# Autodesk Inventor assembly: axis5_6  compact
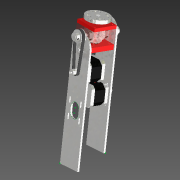
[picture p0: Inventor's stored thumbnail of the model, 180x180]
Saved by Autodesk Inventor 2020 (Build 240168000, 168)
## iProperties
Created: 2020-05-15
Part Number: axis5_6  compact
Document SubType Name: Assembly
Designer: stefa
Author: stefa
## Documents named in this file (9)
- D:\github_gedeeld\BeerMinder\3D-model\axis5_6\axis5_6  compact.iam
- D:\github_gedeeld\BeerMinder\3D-model\pulleys\GT2 Timing Pulley 36T - 8mm as.ipt
- D:\github_gedeeld\BeerMinder\3D-model\stepper motors\42BYG Stepper Motor.ipt
- D:\github_gedeeld\BeerMinder\3D-model\pulleys\GT2 Pulley 16T - 5mm as.ipt
- D:\github_gedeeld\BeerMinder\3D-model\axis5_6\bovenarm - links.ipt
- D:\github_gedeeld\BeerMinder\3D-model\bearings\lager 8mm - buiten 14 (sven 2 stuks).ipt
- D:\github_gedeeld\BeerMinder\3D-model\axis5_6\differential gearbox compact.iam
- D:\github_gedeeld\BeerMinder\3D-model\pulleys\tandriem32Tnaar16T_lengte280.ipt
- D:\github_gedeeld\BeerMinder\3D-model\pulleys\tandriem32Tnaar16T_lengte188.ipt
## Components (13 placed, 8 different names)
1. tandriem32Tnaar16T_lengte280:1 — Mate:57, Mate:58, Mate:106, Mate:107
2. tandriem32Tnaar16T_lengte188:1 — Mate:60, Mate:89, Mate:94, Mate:100
3. 42BYG Stepper Motor:2 — Mate:96, Mate:108, Tangent:120, Tangent:121
4. bovenarm - links:1 — Angle:3, Flush:6, Mate:96, Mate:109, Mate:113, Flush:14, Mate:118, Tangent:120, Tangent:121
5. GT2 Timing Pulley 36T - 8mm as:6 — Mate:57, Mate:58, Mate:115
6. GT2 Timing Pulley 36T - 8mm as:7 — Mate:60, Mate:100, Mate:114
7. bovenarm - links:2 — Flush:6, Mate:99, Mate:102, Flush:10, Mate:103, Mate:104, Mate:105, Mate:112, Flush:13, Mate:117
8. GT2 Pulley 16T - 5mm as:2 — Mate:89, Mate:94, Mate:101, Mate:102
9. GT2 Pulley 16T - 5mm as:3 — Mate:106, Mate:107, Mate:108, Mate:109
10. 42BYG Stepper Motor:3 — Mate:99, Mate:101, Flush:10
11. lager 8mm - buiten 14 (sven 2 stuks):1 — Mate:112, Flush:13
12. lager 8mm - buiten 14 (sven 2 stuks):2 — Mate:113, Flush:14, Mate:116
13. differential gearbox compact:1 [sub-assembly] — Mate:114, Mate:115, Mate:116, Mate:117, Mate:118
## Relationships (31: Mate 24, Flush 4, Tangent 2, Angle 1)
- Angle:3 (0 deg): bovenarm - links:1
- Mate:57 (0.5 mm): tandriem32Tnaar16T_lengte280:1 ↔ GT2 Timing Pulley 36T - 8mm as:6
- Mate:58: tandriem32Tnaar16T_lengte280:1 ↔ GT2 Timing Pulley 36T - 8mm as:6
- Mate:60 (0.5 mm): tandriem32Tnaar16T_lengte188:1 ↔ GT2 Timing Pulley 36T - 8mm as:7
- Flush:6: bovenarm - links:1 ↔ bovenarm - links:2
- Mate:89 (0.5 mm): tandriem32Tnaar16T_lengte188:1 ↔ GT2 Pulley 16T - 5mm as:2
- Mate:94: tandriem32Tnaar16T_lengte188:1 ↔ GT2 Pulley 16T - 5mm as:2
- Mate:96: 42BYG Stepper Motor:2 ↔ bovenarm - links:1
- Mate:99: bovenarm - links:2 ↔ 42BYG Stepper Motor:3
- Mate:100: tandriem32Tnaar16T_lengte188:1 ↔ GT2 Timing Pulley 36T - 8mm as:7
- Mate:101: GT2 Pulley 16T - 5mm as:2 ↔ 42BYG Stepper Motor:3
- Mate:102 (2 mm): bovenarm - links:2 ↔ GT2 Pulley 16T - 5mm as:2
- Flush:10 (-6.55 mm): bovenarm - links:2 ↔ 42BYG Stepper Motor:3
- Mate:103: bovenarm - links:2
- Mate:104: bovenarm - links:2
- Mate:105: bovenarm - links:2
- Mate:106: tandriem32Tnaar16T_lengte280:1 ↔ GT2 Pulley 16T - 5mm as:3
- Mate:107 (0.5 mm): tandriem32Tnaar16T_lengte280:1 ↔ GT2 Pulley 16T - 5mm as:3
- Mate:108: 42BYG Stepper Motor:2 ↔ GT2 Pulley 16T - 5mm as:3
- Mate:109 (2 mm): bovenarm - links:1 ↔ GT2 Pulley 16T - 5mm as:3
- Mate:112: bovenarm - links:2 ↔ lager 8mm - buiten 14 (sven 2 stuks):1
- Flush:13: bovenarm - links:2 ↔ lager 8mm - buiten 14 (sven 2 stuks):1
- Mate:113: bovenarm - links:1 ↔ lager 8mm - buiten 14 (sven 2 stuks):2
- Flush:14: bovenarm - links:1 ↔ lager 8mm - buiten 14 (sven 2 stuks):2
- Mate:114: GT2 Timing Pulley 36T - 8mm as:7 ↔ differential gearbox compact:1
- Mate:115: GT2 Timing Pulley 36T - 8mm as:6 ↔ differential gearbox compact:1
- Mate:116: lager 8mm - buiten 14 (sven 2 stuks):2 ↔ differential gearbox compact:1
- Mate:117 (1 mm): bovenarm - links:2 ↔ differential gearbox compact:1
- Mate:118 (1 mm): bovenarm - links:1 ↔ differential gearbox compact:1
- Tangent:120 (0.3 mm): 42BYG Stepper Motor:2 ↔ bovenarm - links:1
- Tangent:121 (0.3 mm): 42BYG Stepper Motor:2 ↔ bovenarm - links:1
